# Autodesk Inventor assembly: Carcasa SAV
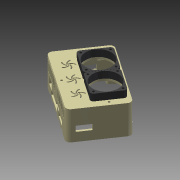
[picture p0: Inventor's stored thumbnail of the model, 180x180]
Saved by Autodesk Inventor 2014 (Build 180170000, 170)
## iProperties
Created: 2014-09-12
Part Number: Carcasa SAV
Document SubType Name: Assembly
Designer: Rubén
Author: Rubén
## Documents named in this file (4)
- C:\Users\Rubén\Desktop\Mis diseños\Prusa i3 Steel parts\SAV case\SAV case (V1).iam
- C:\Users\Rubén\Desktop\Mis diseños\Prusa i3 Steel parts\SAV case\SAV case cover (V1).ipt
- C:\Users\Rubén\Desktop\Mis diseños\Prusa i3 Steel parts\SAV case\Fan 4x4.ipt
- C:\Users\Rubén\Desktop\Mis diseños\Prusa i3 Steel parts\SAV case\SAV case (V1).ipt
## Components (4 placed, 3 different names)
1. SAV case (V1):1 — Mate:1, Mate:2, Mate:3
2. SAV case cover (V1):1 — Mate:1, Mate:2, Mate:3, Mate:4, Mate:5, Mate:6, Mate:7, Mate:8, Mate:9
3. Fan 4x4:1 — Mate:4, Mate:6, Mate:8
4. Fan 4x4:2 — Mate:5, Mate:7, Mate:9
## Relationships (9: Mate 9)
- Mate:1: SAV case (V1):1 ↔ SAV case cover (V1):1
- Mate:2: SAV case (V1):1 ↔ SAV case cover (V1):1
- Mate:3: SAV case (V1):1 ↔ SAV case cover (V1):1
- Mate:4: SAV case cover (V1):1 ↔ Fan 4x4:1
- Mate:5: SAV case cover (V1):1 ↔ Fan 4x4:2
- Mate:6: SAV case cover (V1):1 ↔ Fan 4x4:1
- Mate:7: SAV case cover (V1):1 ↔ Fan 4x4:2
- Mate:8: SAV case cover (V1):1 ↔ Fan 4x4:1
- Mate:9: SAV case cover (V1):1 ↔ Fan 4x4:2
